# Autodesk Inventor assembly: BodyV4
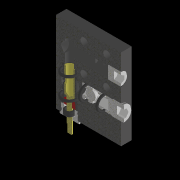
[picture p0: Inventor's stored thumbnail of the model, 180x180]
Saved by Autodesk Inventor 2021 (Build 250183000, 183)
## iProperties
Created: 2024-03-17
Part Number: BodyV4
Document SubType Name: Assembly
Designer: top10
Author: top10
## Documents named in this file (6)
- D:\Files\Graduation Project\V4_manfoulid\Workspaces\Workspace\BodyV4.iam
- D:\Files\Graduation Project\V4_manfoulid\Workspaces\Workspace\Val_BodV4.ipt
- D:\Files\Graduation Project\V4_manfoulid\Workspaces\Workspace\R_nozzle\rotarynozzle.iam
- D:\Files\Graduation Project\V4_manfoulid\Workspaces\Workspace\CheckBall.iam
- D:\Files\Graduation Project\V4_manfoulid\Workspaces\Workspace\M10_HEX.ipt
- D:\Files\Graduation Project\V4_manfoulid\Workspaces\Workspace\M12_HEX.ipt
## Components (5 placed, 5 different names)
1. Val_BodV4:1 — Flush:1, Flush:2, Flush:3, Mate:1, Mate:2, Mate:3, Mate:7, Mate:8, Flush:4
2. rotarynozzle:1 [sub-assembly] — Mate:1, Mate:2, Mate:3
3. CheckBall:1 [sub-assembly] — Mate:9
4. M10_HEX:1 — Mate:7, Flush:4
5. M12_HEX:1 — Mate:8, Mate:9
## Relationships (12: Mate 8, Flush 4)
- Flush:1: Val_BodV4:1
- Flush:2: Val_BodV4:1
- Flush:3: Val_BodV4:1
- Mate:1 (20 mm): Val_BodV4:1 ↔ rotarynozzle:1
- Mate:2: Val_BodV4:1 ↔ rotarynozzle:1
- Mate:3: Val_BodV4:1 ↔ rotarynozzle:1
- [Mate]: Val_BodV4:1 ↔ CheckBall:1
- [Mate]: Val_BodV4:1 ↔ CheckBall:1
- Mate:7: Val_BodV4:1 ↔ M10_HEX:1
- Mate:8: Val_BodV4:1 ↔ M12_HEX:1
- Flush:4: Val_BodV4:1 ↔ M10_HEX:1
- Mate:9: CheckBall:1 ↔ M12_HEX:1
